# Autodesk Inventor assembly: TH1-002_CAM1
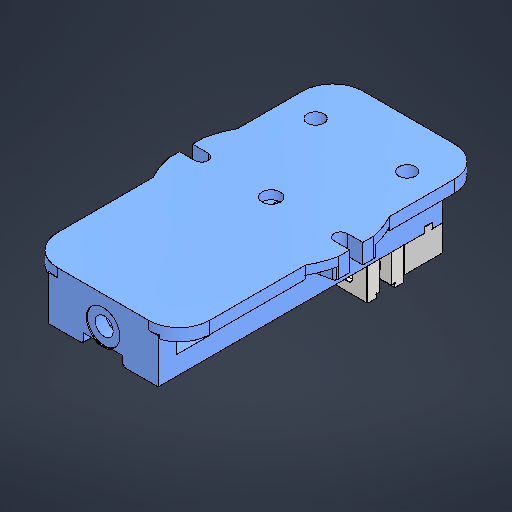
[picture p0: Inventor's stored thumbnail of the model, 512x512]
Saved by Autodesk Inventor 2025.3 (Build 293356000, 356)
## iProperties
Created: 2025-03-10
Part Number: TH1-002_CAM1
Document SubType Name: Assembly
Designer: fablabadmin
Author: fablabadmin
## Documents named in this file (7)
- C:\Users\fablabadmin\Documents\_Benjamin_S\_3dCAD\HHVerkstad\ToolHolder1\_TH1-002_CAM\TH1-002_CAM1.iam
- C:\Users\fablabadmin\Documents\_Benjamin_S\_3dCAD\_Config\KemmlerVise\OP1-KemmlerVise.iam
- C:\Users\fablabadmin\Documents\_Benjamin_S\_3dCAD\_Config\KemmlerVise\OP2-KemmlerVise.iam
- C:\Users\fablabadmin\Documents\_Benjamin_S\_3dCAD\HHVerkstad\ToolHolder1\TH1-002.ipt
- C:\Users\fablabadmin\Documents\_Benjamin_S\_3dCAD\HHVerkstad\ToolHolder1\_TH1-002_CAM\OP1Stock.ipt
- C:\Users\fablabadmin\Documents\Inventor\Content Center Files\R2024\en-US\SteppedJaw\JawSTD-Aluminum 6061-SteppedJaw-Steel, Wrought.ipt
- C:\Users\fablabadmin\Documents\_Benjamin_S\_3dCAD\_Config\_CAM_SIM\FixtureParts\parallels3mm.xlsx
## Components (9 placed, 5 different names)
1. TH1-002:1 — Mate:4, Symmetry:1, Flush:3, Symmetry:2, Mate:6, Flush:4, Mate:26
2. TH1-002:2 — Mate:5, Symmetry:1, Flush:3, Symmetry:2, Mate:6, Mate:14, Mate:27, Mate:28, Mate:29, Angle:1
3. OP1Stock:1 — Flush:4, Flush:5, Flush:6, Mate:20, Mate:21, Mate:22
4. SteppedJaw JawSTD-Aluminum 6061:2 — Mate:18, Flush:9, Mate:21
5. SteppedJaw JawSTD-Aluminum 6061:1 — Mate:17, Flush:8, Flush:9, Mate:19, Mate:20, Mate:22
6. OP1-KemmlerVise:1 [sub-assembly] — Flush:7, Mate:17, Mate:18, Flush:8, Mate:19
7. SteppedJaw JawSTD-Aluminum 6061:3 — Mate:23, Flush:10, Flush:11, Mate:25, Mate:26
8. SteppedJaw JawSTD-Aluminum 6061:4 — Mate:24, Flush:11, Mate:27
9. OP2-KemmlerVise:1 [sub-assembly] — Mate:14, Mate:16, Mate:23, Mate:24, Flush:10, Mate:25, Mate:33
## Relationships (35: Mate 23, Flush 9, Symmetry 2, Angle 1)
- Mate:4: TH1-002:1
- Mate:5: TH1-002:2
- Symmetry:1: TH1-002:1 ↔ TH1-002:2
- Flush:3: TH1-002:1 ↔ TH1-002:2
- Symmetry:2: TH1-002:1 ↔ TH1-002:2
- Mate:6 (8 mm): TH1-002:1 ↔ TH1-002:2
- Flush:4 (-0.5 mm): TH1-002:1 ↔ OP1Stock:1
- Flush:5: OP1Stock:1
- Flush:6: OP1Stock:1
- Flush:7: OP1-KemmlerVise:1
- Mate:14 (35 mm): TH1-002:2 ↔ OP2-KemmlerVise:1
- Mate:16: OP2-KemmlerVise:1
- Mate:17: SteppedJaw JawSTD-Aluminum 6061:1 ↔ OP1-KemmlerVise:1
- Mate:18: SteppedJaw JawSTD-Aluminum 6061:2 ↔ OP1-KemmlerVise:1
- Flush:8: SteppedJaw JawSTD-Aluminum 6061:1 ↔ OP1-KemmlerVise:1
- Flush:9: SteppedJaw JawSTD-Aluminum 6061:2 ↔ SteppedJaw JawSTD-Aluminum 6061:1
- Mate:19: SteppedJaw JawSTD-Aluminum 6061:1 ↔ OP1-KemmlerVise:1
- Mate:20: OP1Stock:1 ↔ SteppedJaw JawSTD-Aluminum 6061:1
- Mate:21: OP1Stock:1 ↔ SteppedJaw JawSTD-Aluminum 6061:2
- Mate:22: OP1Stock:1 ↔ SteppedJaw JawSTD-Aluminum 6061:1
- Mate:23: SteppedJaw JawSTD-Aluminum 6061:3 ↔ OP2-KemmlerVise:1
- Mate:24: SteppedJaw JawSTD-Aluminum 6061:4 ↔ OP2-KemmlerVise:1
- Flush:10: SteppedJaw JawSTD-Aluminum 6061:3 ↔ OP2-KemmlerVise:1
- Flush:11: SteppedJaw JawSTD-Aluminum 6061:3 ↔ SteppedJaw JawSTD-Aluminum 6061:4
- Mate:25: SteppedJaw JawSTD-Aluminum 6061:3 ↔ OP2-KemmlerVise:1
- Mate:26: TH1-002:1 ↔ SteppedJaw JawSTD-Aluminum 6061:3
- Mate:27: TH1-002:2 ↔ SteppedJaw JawSTD-Aluminum 6061:4
- Mate:28: TH1-002:2
- Mate:29: TH1-002:2
- Mate:30
- Mate:31
- Mate:32
- Angle:1 (0 deg): TH1-002:2
- Mate:33: OP2-KemmlerVise:1
- Mate:34
## Named parameters: PRL13 = 13 mm, PRL16 = 16 mm, PRL19 = 19 mm, PRL22 = 22 mm, PRL28 = 28 mm, PRL31 = 31 mm, PRL35 = 35 mm, PRL38 = 38 mm, PRL41 = 41 mm
